# Autodesk Inventor assembly: strojniSklop
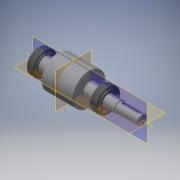
[picture p0: Inventor's stored thumbnail of the model, 180x180]
Saved by Autodesk Inventor 2018 (Build 220112000, 112)
## iProperties
Created: 2018-05-05
Part Number: strojniSklop
Document SubType Name: Assembly
Designer: Kristijan
Author: Kristijan
## Documents named in this file (3)
- C:\Users\krist\Dropbox (Personal)\PolitehnikaPula\4 semestar\Elementi strojeva 2\projektniZadatak\strojniSklop.iam
- C:\Users\krist\Dropbox (Personal)\PolitehnikaPula\4 semestar\Elementi strojeva 2\projektniZadatak\vratilo.ipt
- C:\Users\krist\Dropbox (Personal)\PolitehnikaPula\4 semestar\Elementi strojeva 2\projektniZadatak\6205.iam
## Components (3 placed, 2 different names)
1. vratilo:1 — Mate:1, Mate:2, Mate:3, Mate:4
2. 6205:1 [sub-assembly] — Mate:1, Mate:2
3. 6205:2 [sub-assembly] — Mate:3, Mate:4
## Relationships (4: Mate 4)
- Mate:1: vratilo:1 ↔ 6205:1
- Mate:2: vratilo:1 ↔ 6205:1
- Mate:3: vratilo:1 ↔ 6205:2
- Mate:4: vratilo:1 ↔ 6205:2
